# Autodesk Inventor assembly: Esp_pcb
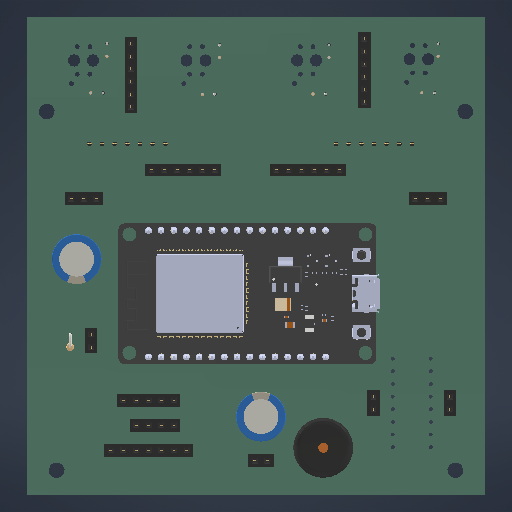
[picture p0: Inventor's stored thumbnail of the model, 512x512]
Saved by Autodesk Inventor 2026 (Build 300175000, 175)
## iProperties
Company: Kicad
Created: 2025-11-05
Part Number: Esp_pcb
Description: KiCad electronic assembly
Document SubType Name: Assembly
Designer: pregu
Authority: Unknown
Sending System: KiCad to STEP converter
Preprocessor: Open CASCADE STEP processor 7.9
Title: esp-car.step
Author: Pcbnew
## Documents named in this file (13)
- C:\Users\pregu\OneDrive\Documentos\Carro 8.5\Esp_pcb.iam
- C:\Users\pregu\Downloads\esp-car-newvember\esp-car-newvember\PinSocket_1x04_P2.54mm_Vertical.ipt
- C:\Users\pregu\Downloads\esp-car-newvember\esp-car-newvember\PinSocket_1x02_P2.54mm_Vertical.ipt
- C:\Users\pregu\Downloads\esp-car-newvember\esp-car-newvember\PinSocket_1x15_P2.54mm_Vertical.ipt
- C:\Users\pregu\Downloads\esp-car-newvember\esp-car-newvember\PinSocket_1x03_P2.54mm_Vertical.ipt
- C:\Users\pregu\Downloads\esp-car-newvember\esp-car-newvember\PinSocket_1x06_P2.54mm_Vertical.ipt
- C:\Users\pregu\Downloads\esp-car-newvember\esp-car-newvember\PinSocket_1x05_P2.54mm_Vertical.ipt
- C:\Users\pregu\Downloads\esp-car-newvember\esp-car-newvember\CP_Radial_D10.0mm_P3.50mm.ipt
- C:\Users\pregu\Downloads\esp-car-newvember\esp-car-newvember\Buzzer_12x9.5RM7.6.ipt
- C:\Users\pregu\Downloads\esp-car-newvember\esp-car-newvember\PinSocket_1x07_P2.54mm_Vertical.ipt
- C:\Users\pregu\Downloads\esp-car-newvember\esp-car-newvember\R_Axial_DIN0204_L3.6mm_D1.6mm_P2.54mm_Vertical.ipt
- C:\Users\pregu\Downloads\esp-car-newvember\esp-car-newvember\esp-car_PCB.ipt
- C:\Users\pregu\Downloads\Soccer_Pedro\ESP32-DEVKIT-V1-30-PIN.ipt
## Components (31 placed, 31 different names)
1. 1
2. 2
3. 3 — Coincidente:1, Coincidente:2
4. 4
5. 5
6. 6
7. 7
8. 8
9. 9
10. 10
11. 11
12. 12
13. 13
14. 14
15. 15
16. 16
17. 17
18. 18
19. 19
20. 20
21. 21
22. 22
23. 23
24. 24
25. 25
26. 26
27. 27
28. 28
29. 29
30. 30
31. ESP32-DEVKIT-V1-30-PIN:1 — Coincidente:1, Coincidente:2
## Relationships (2: Mate 2)
- Coincidente:1 [Mate]: 3 ↔ ESP32-DEVKIT-V1-30-PIN:1
- Coincidente:2 [Mate]: 3 ↔ ESP32-DEVKIT-V1-30-PIN:1
